# Autodesk Inventor assembly: bottom_chassis
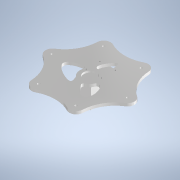
[picture p0: Inventor's stored thumbnail of the model, 180x180]
Saved by Autodesk Inventor 2020.2 (Build 242310000, 310)
## iProperties
Created: 2020-11-22
Part Number: bottom_chassis
Document SubType Name: Assembly
Designer: mazzo
Author: mazzo
## Documents named in this file (3)
- D:\Documenti\università\Progetto Meccanica dei Robot\assembled in urdf\bottom_chassis.iam
- D:\Documenti\università\Progetto Meccanica dei Robot\meccanica\parti autodesk\V6\V6 Luca\bottom_down_chassis.ipt
- D:\Documenti\università\Progetto Meccanica dei Robot\meccanica\parti autodesk\V6\V6 Luca\Motore1.ipt
## Components (2 placed, 2 different names)
1. bottom_down_chassis:1 — Coincidente:1, Allineato:1, Coincidente:2, Coincidente:3, Coincidente:4
2. Motore1:1 — Coincidente:2, Coincidente:3, Angolo:1
## Relationships (6: Mate 4, Flush 1, Angle 1)
- Coincidente:1 [Mate]: bottom_down_chassis:1
- Allineato:1 [Flush]: bottom_down_chassis:1
- Coincidente:2 [Mate]: bottom_down_chassis:1 ↔ Motore1:1
- Coincidente:3 [Mate]: bottom_down_chassis:1 ↔ Motore1:1
- Coincidente:4 [Mate]: bottom_down_chassis:1
- Angolo:1 [Angle] (0 deg): Motore1:1
